# Autodesk Inventor assembly: MotorLeft
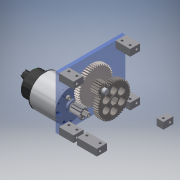
[picture p0: Inventor's stored thumbnail of the model, 180x180]
Saved by Autodesk Inventor 2019 (Build 230136000, 136)
## iProperties
Created: 2020-02-28
Part Number: MotorLeft
Document SubType Name: Assembly
Designer: james
Author: james
## Documents named in this file (14)
- F:\JimsRobot\FIRSTRobots\Design\TornadoPlatypus\MotorLeft.iam
- F:\JimsRobot\FIRSTRobots\Design\TornadoPlatypus\InsideMotorPlate.ipt
- F:\JimsRobot\FIRSTRobots\Design\Library\CTR\Falcon\217-6515 20191025.iam
- F:\JimsRobot\FIRSTRobots\Design\Library\AndyMark\FR6ZZ Bearing.ipt
- F:\JimsRobot\FIRSTRobots\Design\TornadoPlatypus\MotorSpacerBlock.ipt
- F:\JimsRobot\FIRSTRobots\Design\Library\AndyMark\Toughbox d07.ipt
- F:\JimsRobot\FIRSTRobots\Design\Library\AndyMark\6 HiGrip Asm Rev II.iam
- F:\JimsRobot\FIRSTRobots\Design\TornadoPlatypus\MotorSpacerBlock2.ipt
- F:\JimsRobot\FIRSTRobots\Design\TornadoPlatypus\MotorSpacerBlock3.ipt
- F:\JimsRobot\FIRSTRobots\Design\Library\CTR\10T_20DP_FALCON.ipt
- F:\JimsRobot\FIRSTRobots\Design\Library\Fasteners\Size-10-32\HexCap-1.ipt
- F:\JimsRobot\FIRSTRobots\Design\Library\AndyMark\am-0149 50T 20dp 375hex REV2.ipt
- F:\JimsRobot\FIRSTRobots\Design\Library\AndyMark\am-0747 16t 20dp 375h with teeth.ipt
- F:\JimsRobot\FIRSTRobots\Design\Library\AndyMark\am-0184 48T 500in Hex Bore Gear REV2 (1).ipt
## Components (22 placed, 13 different names)
1. InsideMotorPlate:1 — Mate:1, Mate:2, Mate:3, Mate:5, Mate:6, Mate:7, Mate:8, Mate:9, Mate:10, Mate:11, Flush:1, Mate:12, Flush:2, Mate:13, Flush:3, Mate:14, Flush:4, Mate:21, Mate:22, Mate:42, Mate:44, Mate:45, Mate:46, Mate:50
2. 217-6515 20191025:1 [sub-assembly] — Mate:1, Mate:2, Mate:3, Mate:43
3. FR6ZZ Bearing:1 — Mate:5, Mate:6, Mate:15, Flush:5, Mate:48
4. MotorSpacerBlock:1 — Mate:9, Mate:13, Flush:3, Mate:26, Mate:28
5. MotorSpacerBlock:2 — Mate:7, Mate:12, Flush:2
6. MotorSpacerBlock:3 — Mate:10, Mate:11, Flush:1
7. MotorSpacerBlock:4 — Mate:8, Mate:14, Flush:4, Mate:27
8. Toughbox d07:1 — Mate:15, Flush:5, Mate:49, Mate:52
9. FR6ZZ Bearing:2 — Mate:21, Mate:22, Mate:54
10. InsideMotorPlate:2 — Mate:26, Mate:27, Mate:28, Mate:29, Mate:30, Mate:31, Mate:32, Mate:33, Flush:6, Mate:34, Flush:7
11. 6 HiGrip Asm Rev II:1 [sub-assembly] — Mate:29, Mate:30
12. MotorSpacerBlock2:1 — Mate:32, Mate:34, Flush:7, Mate:35, Mate:37
13. MotorSpacerBlock2:2 — Mate:31, Mate:33, Flush:6, Mate:36
14. InsideMotorPlate:3 — Mate:35, Mate:36, Mate:37, Mate:38, Mate:39, Flush:8, Mate:40, Mate:41, Flush:9
15. MotorSpacerBlock3:1 — Mate:38, Mate:39, Flush:8
16. MotorSpacerBlock3:2 — Mate:40, Mate:41, Flush:9
17. 10T_20DP_FALCON:1 — Mate:42, Mate:43
18. HexCap-1:1 — Mate:44, Mate:50
19. HexCap-1:2 — Mate:45, Mate:46
20. am-0149 50T 20dp 375hex REV2:1 — Mate:48, Mate:49, Mate:51, Mate:53
21. am-0747 16t 20dp 375h with teeth:1 — Mate:51, Mate:52
22. am-0184 48T 500in Hex Bore Gear REV2 (1):1 — Mate:53, Mate:54
## Relationships (53: Mate 44, Flush 9)
- Mate:1: InsideMotorPlate:1 ↔ 217-6515 20191025:1
- Mate:2: InsideMotorPlate:1 ↔ 217-6515 20191025:1
- Mate:3: InsideMotorPlate:1 ↔ 217-6515 20191025:1
- Mate:5: InsideMotorPlate:1 ↔ FR6ZZ Bearing:1
- Mate:6: InsideMotorPlate:1 ↔ FR6ZZ Bearing:1
- Mate:7: InsideMotorPlate:1 ↔ MotorSpacerBlock:2
- Mate:8: InsideMotorPlate:1 ↔ MotorSpacerBlock:4
- Mate:9: InsideMotorPlate:1 ↔ MotorSpacerBlock:1
- Mate:10: InsideMotorPlate:1 ↔ MotorSpacerBlock:3
- Mate:11: InsideMotorPlate:1 ↔ MotorSpacerBlock:3
- Flush:1: InsideMotorPlate:1 ↔ MotorSpacerBlock:3
- Mate:12: InsideMotorPlate:1 ↔ MotorSpacerBlock:2
- Flush:2: InsideMotorPlate:1 ↔ MotorSpacerBlock:2
- Mate:13: InsideMotorPlate:1 ↔ MotorSpacerBlock:1
- Flush:3: InsideMotorPlate:1 ↔ MotorSpacerBlock:1
- Mate:14: InsideMotorPlate:1 ↔ MotorSpacerBlock:4
- Flush:4: InsideMotorPlate:1 ↔ MotorSpacerBlock:4
- Mate:15: FR6ZZ Bearing:1 ↔ Toughbox d07:1
- Flush:5: FR6ZZ Bearing:1 ↔ Toughbox d07:1
- Mate:21: InsideMotorPlate:1 ↔ FR6ZZ Bearing:2
- Mate:22: InsideMotorPlate:1 ↔ FR6ZZ Bearing:2
- Mate:26: MotorSpacerBlock:1 ↔ InsideMotorPlate:2
- Mate:27: MotorSpacerBlock:4 ↔ InsideMotorPlate:2
- Mate:28: MotorSpacerBlock:1 ↔ InsideMotorPlate:2
- Mate:29: InsideMotorPlate:2 ↔ 6 HiGrip Asm Rev II:1
- Mate:30: InsideMotorPlate:2 ↔ 6 HiGrip Asm Rev II:1
- Mate:31: InsideMotorPlate:2 ↔ MotorSpacerBlock2:2
- Mate:32: InsideMotorPlate:2 ↔ MotorSpacerBlock2:1
- Mate:33: InsideMotorPlate:2 ↔ MotorSpacerBlock2:2
- Flush:6: InsideMotorPlate:2 ↔ MotorSpacerBlock2:2
- Mate:34: InsideMotorPlate:2 ↔ MotorSpacerBlock2:1
- Flush:7: InsideMotorPlate:2 ↔ MotorSpacerBlock2:1
- Mate:35: MotorSpacerBlock2:1 ↔ InsideMotorPlate:3
- Mate:36: MotorSpacerBlock2:2 ↔ InsideMotorPlate:3
- Mate:37: MotorSpacerBlock2:1 ↔ InsideMotorPlate:3
- Mate:38: InsideMotorPlate:3 ↔ MotorSpacerBlock3:1
- Mate:39: InsideMotorPlate:3 ↔ MotorSpacerBlock3:1
- Flush:8: InsideMotorPlate:3 ↔ MotorSpacerBlock3:1
- Mate:40: InsideMotorPlate:3 ↔ MotorSpacerBlock3:2
- Mate:41: InsideMotorPlate:3 ↔ MotorSpacerBlock3:2
- Flush:9: InsideMotorPlate:3 ↔ MotorSpacerBlock3:2
- Mate:42: InsideMotorPlate:1 ↔ 10T_20DP_FALCON:1
- Mate:43: 217-6515 20191025:1 ↔ 10T_20DP_FALCON:1
- Mate:44: InsideMotorPlate:1 ↔ HexCap-1:1
- Mate:45: InsideMotorPlate:1 ↔ HexCap-1:2
- Mate:46: InsideMotorPlate:1 ↔ HexCap-1:2
- Mate:48: FR6ZZ Bearing:1 ↔ am-0149 50T 20dp 375hex REV2:1
- Mate:49: Toughbox d07:1 ↔ am-0149 50T 20dp 375hex REV2:1
- Mate:50: InsideMotorPlate:1 ↔ HexCap-1:1
- Mate:51: am-0149 50T 20dp 375hex REV2:1 ↔ am-0747 16t 20dp 375h with teeth:1
- Mate:52: Toughbox d07:1 ↔ am-0747 16t 20dp 375h with teeth:1
- Mate:53: am-0149 50T 20dp 375hex REV2:1 ↔ am-0184 48T 500in Hex Bore Gear REV2 (1):1
- Mate:54: FR6ZZ Bearing:2 ↔ am-0184 48T 500in Hex Bore Gear REV2 (1):1
